# Autodesk Inventor assembly: Assembly2
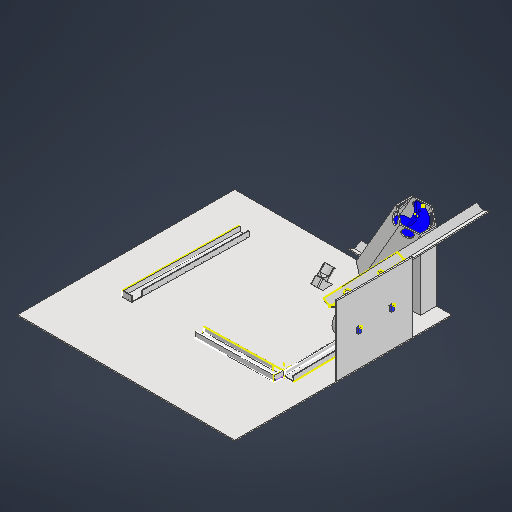
[picture p0: Inventor's stored thumbnail of the model, 512x512]
Saved by Autodesk Inventor 2026.1 (Build 301233020, 233B)
## iProperties
Created: 2026-05-02
Part Number: Assembly2
Document SubType Name: Assembly
Designer: hp
Author: hp
## Documents named in this file (12)
- C:\Users\hp\OneDrive\Documents\Inventor\BOM\Assembly2.iam
- C:\Users\hp\OneDrive\Documents\Inventor\BOM\base.ipt
- C:\Users\hp\OneDrive\Documents\Inventor\BOM\LIFTER SUPPORT.ipt
- C:\Users\hp\OneDrive\Documents\Inventor\BOM\Lifting.iam
- C:\Users\hp\OneDrive\Documents\Inventor\BOM\rail 3.ipt
- C:\Users\hp\OneDrive\Documents\Inventor\BOM\rail 2.ipt
- C:\Users\hp\OneDrive\Documents\Inventor\BOM\subsystem sorter finale.iam
- C:\Users\hp\OneDrive\Documents\Inventor\BOM\medium yellow ball.ipt
- C:\Users\hp\OneDrive\Documents\Inventor\BOM\rail 11.ipt
- C:\Users\hp\OneDrive\Documents\Inventor\BOM\rail 22.ipt
- C:\Users\hp\OneDrive\Documents\Inventor\BOM\rail 33.ipt
- C:\Users\hp\OneDrive\Documents\Inventor\BOM\Shooter.ipt
## Components (11 placed, 11 different names)
1. base:1 — Mate:6, Mate:14, Mate:15, Mate:16, Mate:17, Mate:18, Mate:19
2. LIFTER SUPPORT:1 — Mate:3, Mate:4, Mate:5, Mate:6, Mate:11, Mate:14, Mate:15, Mate:16, Mate:23
3. Lifting:1 [sub-assembly] — Mate:3, Mate:4, Mate:5, Mate:11
4. rail 3:1
5. subsystem sorter finale:1 [sub-assembly] — Mate:17, Mate:18, Mate:19, Mate:20, Mate:21, Mate:22
6. rail 2:2 — Mate:20, Mate:21, Mate:22, Mate:23
7. medium yellow ball:1
8. rail 11:1
9. rail 22:1
10. rail 33:1
11. Shooter:1
## Relationships (15: Mate 15)
- Mate:3: LIFTER SUPPORT:1 ↔ Lifting:1
- Mate:4: LIFTER SUPPORT:1 ↔ Lifting:1
- Mate:5: LIFTER SUPPORT:1 ↔ Lifting:1
- Mate:6: base:1 ↔ LIFTER SUPPORT:1
- Mate:11: LIFTER SUPPORT:1 ↔ Lifting:1
- Mate:14: base:1 ↔ LIFTER SUPPORT:1
- Mate:15: base:1 ↔ LIFTER SUPPORT:1
- Mate:16: base:1 ↔ LIFTER SUPPORT:1
- Mate:17: base:1 ↔ subsystem sorter finale:1
- Mate:18: base:1 ↔ subsystem sorter finale:1
- Mate:19: base:1 ↔ subsystem sorter finale:1
- Mate:20: subsystem sorter finale:1 ↔ rail 2:2
- Mate:21: subsystem sorter finale:1 ↔ rail 2:2
- Mate:22: subsystem sorter finale:1 ↔ rail 2:2
- Mate:23: LIFTER SUPPORT:1 ↔ rail 2:2
